# Autodesk Inventor assembly: Encoder_Mount2
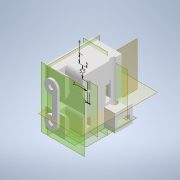
[picture p0: Inventor's stored thumbnail of the model, 180x180]
Saved by Autodesk Inventor 2022 (Build 260153000, 153)
## iProperties
Created: 2024-05-02
Part Number: Encoder_Mount2
Document SubType Name: Assembly
Designer: Gotham City
Author: Gotham City
## Documents named in this file (4)
- E:\inkjet-printer\cad\Encoder_Mount2.iam
- E:\inkjet-printer\cad\Encoder_Mount2.ipt
- E:\inkjet-printer\cad\Encoder_Mount3_Washer.ipt
- E:\inkjet-printer\cad\Encoder_Cable_Clamp.ipt
## Components (3 placed, 3 different names)
1. Encoder_Mount2:1 — Flush:1, Flush:4
2. Encoder_Mount3_Washer:1 — Flush:2, Flush:3
3. Encoder_Cable_Clamp:1 — Flush:4
## Relationships (4: Flush 4)
- Flush:1 (1 mm): Encoder_Mount2:1
- Flush:2: Encoder_Mount3_Washer:1
- Flush:3: Encoder_Mount3_Washer:1
- Flush:4: Encoder_Mount2:1 ↔ Encoder_Cable_Clamp:1
